# Autodesk Inventor assembly: jetsonassem
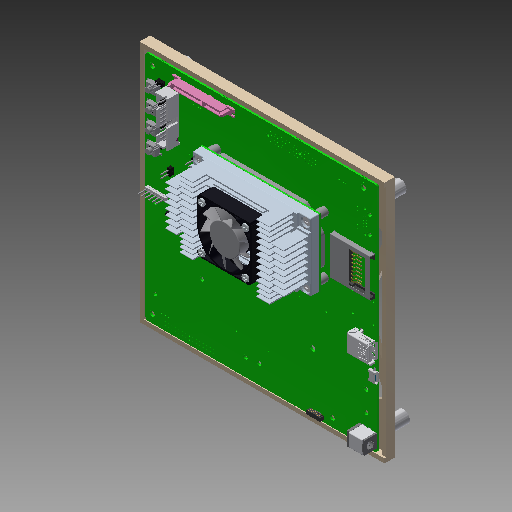
[picture p0: Inventor's stored thumbnail of the model, 512x512]
Saved by Autodesk Inventor 2018 (Build 220112000, 112)
## iProperties
Created: 2018-08-03
Part Number: jetsonassem
Document SubType Name: Assembly
Designer: Cole Tucker
Mass: 185.919 g
Surface Area: 1948.76 cm^2
Volume: 149.836 cm^3
Density: 1.24082 g/cm^3
Author: Cole Tucker
## Documents named in this file (4)
- C:\Users\Cole Tucker\OneDrive\FRC-mxpProject\Cad\ControlCase\Inventor\jetsonassem.iam
- C:\Users\Cole Tucker\OneDrive\FRC-mxpProject\Cad\ControlCase\Inventor\jetson\P2371-top_asm.iam
- C:\Users\Cole Tucker\OneDrive\FRC-mxpProject\Cad\ControlCase\Inventor\jetsonHolder.ipt
- C:\Users\Cole Tucker\OneDrive\FRC-mxpProject\Cad\ControlCase\Inventor\jetsonspacer.ipt
## Components (6 placed, 3 different names)
1. P2371-top_asm:1 [sub-assembly] — Mate:1, Flush:1, Flush:2
2. jetsonHolder:1 — Mate:1, Flush:1, Flush:2, Mate:2, Mate:3, Mate:4, Mate:5, Mate:8, Mate:9, Mate:10, Mate:11
3. jetsonspacer:1 — Mate:5, Mate:8
4. jetsonspacer:2 — Mate:3, Mate:10
5. jetsonspacer:3 — Mate:2, Mate:9
6. jetsonspacer:4 — Mate:4, Mate:11
## Relationships (11: Mate 9, Flush 2)
- Mate:1: P2371-top_asm:1 ↔ jetsonHolder:1
- Flush:1 (5.08 mm): P2371-top_asm:1 ↔ jetsonHolder:1
- Flush:2 (4.064 mm): P2371-top_asm:1 ↔ jetsonHolder:1
- Mate:2: jetsonHolder:1 ↔ jetsonspacer:3
- Mate:3: jetsonHolder:1 ↔ jetsonspacer:2
- Mate:4: jetsonHolder:1 ↔ jetsonspacer:4
- Mate:5: jetsonHolder:1 ↔ jetsonspacer:1
- Mate:8: jetsonHolder:1 ↔ jetsonspacer:1
- Mate:9: jetsonHolder:1 ↔ jetsonspacer:3
- Mate:10: jetsonHolder:1 ↔ jetsonspacer:2
- Mate:11: jetsonHolder:1 ↔ jetsonspacer:4
